# Autodesk Inventor assembly: beercart assembly - mekatronik
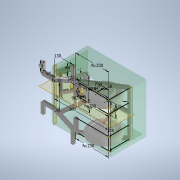
[picture p0: Inventor's stored thumbnail of the model, 180x180]
Saved by Autodesk Inventor 2022.2 (Build 262287000, 287)
## iProperties
_SolveAssemblyDoc: Frame Generator Solve Assembly
_Version: 15.0.0
Created: 2022-03-11
Part Number: beercart assembly - mekatronik
Document SubType Name: Assembly
Designer: foriw
Mass: 10681.4 g
Surface Area: 14312.4 cm^2
Volume: 7244.27 cm^3
Density: 1.47447 g/cm^3
Author: foriw
## Documents named in this file (7)
- C:\Users\foriw\OneDrive\Dokumenter\Inventor\BeerCart - Github - Mekatronik\BeerCart-CAD-Inventor\Workspaces\Workspace\beercart assembly - mekatronik.iam
- C:\Users\foriw\OneDrive\Dokumenter\Inventor\BeerCart - Github - Mekatronik\BeerCart-CAD-Inventor\Workspaces\Workspace\beercart- framwork - baseSketch.ipt
- C:\Users\foriw\OneDrive\Dokumenter\Inventor\BeerCart - Github - Mekatronik\BeerCart-CAD-Inventor\Workspaces\Workspace\beercart assembly - mekatronik\Frame\Frame 1647030135921.iam
- C:\Users\foriw\OneDrive\Dokumenter\Inventor\BeerCart - Github - Mekatronik\BeerCart-CAD-Inventor\Workspaces\Workspace\motor at24v.ipt
- C:\Users\foriw\OneDrive\Dokumenter\Inventor\BeerCart - Github - Mekatronik\BeerCart-CAD-Inventor\Workspaces\Workspace\beer crate.ipt
- C:\Users\foriw\OneDrive\Dokumenter\Inventor\BeerCart - Github - Mekatronik\BeerCart-CAD-Inventor\Workspaces\Workspace\Mekatronik-beerCart\frontwheel frame.ipt
- C:\Users\foriw\OneDrive\Dokumenter\Inventor\BeerCart - Github - Mekatronik\BeerCart-CAD-Inventor\Workspaces\Workspace\motor at24v_MIR.ipt
## Components (6 placed, 6 different names)
1. beercart- framwork - baseSketch:1
2. Frame 1647030135921:1 [sub-assembly] — Flush:3, Insert:2, Insert:3
3. motor at24v:1
4. beer crate:1 — Flush:2, Flush:3
5. frontwheel frame:1
6. motor at24v_MIR:1 — Insert:2, Insert:3
## Relationships (5: Insert 3, Flush 2)
- Flush:2: beer crate:1
- Flush:3: Frame 1647030135921:1 ↔ beer crate:1
- [Insert]: Frame 1647030135921:1 ↔ motor at24v_MIR:1
- Insert:2: Frame 1647030135921:1 ↔ motor at24v_MIR:1
- Insert:3: Frame 1647030135921:1 ↔ motor at24v_MIR:1
